# Autodesk Inventor assembly: GPS_IMUMount
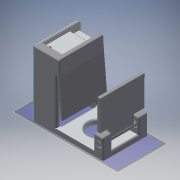
[picture p0: Inventor's stored thumbnail of the model, 180x180]
Saved by Autodesk Inventor 2016 (Build 200138000, 138)
## iProperties
Created: 2016-10-17
Part Number: GPS_IMUMount
Document SubType Name: Assembly
Designer: lachesis
Author: lachesis
## Documents named in this file (3)
- C:\Users\lachesis\git\Swarmathon-Robot\CAD-Files\Parts\GPS_IMUMount\GPS_IMUMount.iam
- C:\Users\lachesis\git\Swarmathon-Robot\CAD-Files\Parts\GPS_IMUMount\GPS_IMUMount.ipt
- C:\Users\lachesis\git\Swarmathon-Robot\CAD-Files\Parts\GPS_IMUMount\GPSDoor.ipt
## Components (2 placed, 2 different names)
1. GPS_IMUMount:1 — Rotational:1, Flush:1
2. GPSDoor:1 — Rotational:1
## Relationships (2: RevoluteJoint 1, Flush 1)
- Rotational:1 [RevoluteJoint]: GPS_IMUMount:1 ↔ GPSDoor:1
- Flush:1 (-19.05 mm): GPS_IMUMount:1
